# Autodesk Inventor assembly: BG401_trajan20_21
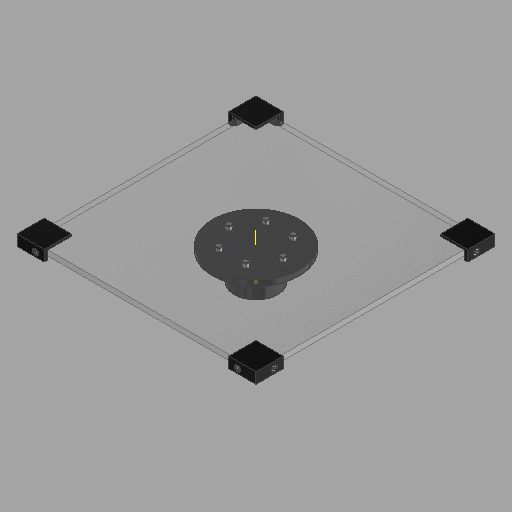
[picture p0: Inventor's stored thumbnail of the model, 512x512]
Saved by Autodesk Inventor 2022.2 (Build 262287000, 287)
## iProperties
Company: HTBLA Kaindorf
RuleStatus: InUse
Created: 2022-08-22
Part Number: BG401_trajan20_21
Project: Zeichenmaschine_v2
Material: Generisch
Description: papierplatte
Document SubType Name: Assembly
Designer: trajan20
AfterDocNew0: iProperties-Editor_aufrufen
Author: jan
Keywords: 2021
## Documents named in this file (6)
- C:\Users\jan\Documents\DrawMachine\DrawMachineConstruction\Projekt\Zeichenmaschine_v2\BG401_trajan20_21_Zeichenmaschine_v2_papierplatte.iam
- C:\Users\jan\Documents\DrawMachine\DrawMachineConstruction\Projekt\Zeichenmaschine_v2\BT403_trajan20_21_Zeichenmaschine_v2_papierplatte_plexi.ipt
- C:\Users\jan\Documents\DrawMachine\DrawMachineConstruction\Projekt\Zeichenmaschine_v2\BT406_trajan20_21_Zeichenmaschine_v2_Ecken.ipt
- C:\Users\jan\Documents\DrawMachine\DrawMachineConstruction\Projekt\Zeichenmaschine_v2\Normteile\de-DE\ISO 4762(2)\ISO 4762 - M3 x 8ISO.ipt
- C:\Users\jan\Documents\DrawMachine\DrawMachineConstruction\Projekt\Zeichenmaschine_v2\BT405_trajan20_21_Zeichenmaschine_v2_zwischenteil_stifte.ipt
- C:\Users\jan\Documents\DrawMachine\DrawMachineConstruction\Projekt\Zeichenmaschine_v2\Normteile\de-DE\ISO 2338(1)\DIN EN ISO 2338 - 5 h8 x 16.ipt
## Components (20 placed, 5 different names)
1. BT403_trajan20_21_Zeichenmaschine_v2_papierplatte_plexi:1 — Passend:1, Passend:2, Passend:3, Passend:7, Passend:8, Passend:9, Passend:10, Passend:11, Passend:12, Passend:13, Passend:14, Passend:15, Passend:28, Passend:29, Passend:30, Passend:31, Passend:32, Passend:33, Passend:34, Passend:35, Passend:36, Passend:37, Passend:38, Passend:39, Passend:40
2. BT406_trajan20_21_Zeichenmaschine_v2_Ecken:1 — Passend:1, Passend:2, Passend:4, Passend:5, Passend:6
3. ISO 4762 M3 x 8:1 — Passend:3, Passend:4
4. ISO 4762 M3 x 8:2 — Passend:5, Passend:6
5. BT406_trajan20_21_Zeichenmaschine_v2_Ecken:2 — Passend:7, Passend:8, Passend:9, Passend:16, Passend:17, Passend:18, Passend:19
6. BT406_trajan20_21_Zeichenmaschine_v2_Ecken:3 — Passend:10, Passend:11, Passend:12, Passend:24, Passend:25, Passend:26, Passend:27
7. BT406_trajan20_21_Zeichenmaschine_v2_Ecken:4 — Passend:13, Passend:14, Passend:15, Passend:20, Passend:21, Passend:22, Passend:23
8. ISO 4762 M3 x 8:3 — Passend:16, Passend:17
9. ISO 4762 M3 x 8:4 — Passend:18, Passend:19
10. ISO 4762 M3 x 8:5 — Passend:20, Passend:21
11. ISO 4762 M3 x 8:6 — Passend:22, Passend:23
12. ISO 4762 M3 x 8:7 — Passend:24, Passend:25
13. ISO 4762 M3 x 8:8 — Passend:26, Passend:27
14. BT405_trajan20_21_Zeichenmaschine_v2_zwischenteil_stifte:1 — Passend:28, Passend:41, Passend:42
15. DIN EN ISO 2338 5 h8 x 16:1 — Passend:29, Passend:30
16. DIN EN ISO 2338 5 h8 x 16:2 — Passend:31, Passend:32, Passend:42
17. DIN EN ISO 2338 5 h8 x 16:3 — Passend:33, Passend:34
18. DIN EN ISO 2338 5 h8 x 16:4 — Passend:35, Passend:36
19. DIN EN ISO 2338 5 h8 x 16:5 — Passend:37, Passend:38, Passend:41
20. DIN EN ISO 2338 5 h8 x 16:6 — Passend:39, Passend:40
## Relationships (42: Mate 42)
- Passend:1 [Mate]: BT403_trajan20_21_Zeichenmaschine_v2_papierplatte_plexi:1 ↔ BT406_trajan20_21_Zeichenmaschine_v2_Ecken:1
- Passend:2 [Mate]: BT403_trajan20_21_Zeichenmaschine_v2_papierplatte_plexi:1 ↔ BT406_trajan20_21_Zeichenmaschine_v2_Ecken:1
- Passend:3 [Mate]: BT403_trajan20_21_Zeichenmaschine_v2_papierplatte_plexi:1 ↔ ISO 4762 M3 x 8:1
- Passend:4 [Mate]: BT406_trajan20_21_Zeichenmaschine_v2_Ecken:1 ↔ ISO 4762 M3 x 8:1
- Passend:5 [Mate]: BT406_trajan20_21_Zeichenmaschine_v2_Ecken:1 ↔ ISO 4762 M3 x 8:2
- Passend:6 [Mate]: BT406_trajan20_21_Zeichenmaschine_v2_Ecken:1 ↔ ISO 4762 M3 x 8:2
- Passend:7 [Mate]: BT403_trajan20_21_Zeichenmaschine_v2_papierplatte_plexi:1 ↔ BT406_trajan20_21_Zeichenmaschine_v2_Ecken:2
- Passend:8 [Mate]: BT403_trajan20_21_Zeichenmaschine_v2_papierplatte_plexi:1 ↔ BT406_trajan20_21_Zeichenmaschine_v2_Ecken:2
- Passend:9 [Mate]: BT403_trajan20_21_Zeichenmaschine_v2_papierplatte_plexi:1 ↔ BT406_trajan20_21_Zeichenmaschine_v2_Ecken:2
- Passend:10 [Mate]: BT403_trajan20_21_Zeichenmaschine_v2_papierplatte_plexi:1 ↔ BT406_trajan20_21_Zeichenmaschine_v2_Ecken:3
- Passend:11 [Mate]: BT403_trajan20_21_Zeichenmaschine_v2_papierplatte_plexi:1 ↔ BT406_trajan20_21_Zeichenmaschine_v2_Ecken:3
- Passend:12 [Mate]: BT403_trajan20_21_Zeichenmaschine_v2_papierplatte_plexi:1 ↔ BT406_trajan20_21_Zeichenmaschine_v2_Ecken:3
- Passend:13 [Mate]: BT403_trajan20_21_Zeichenmaschine_v2_papierplatte_plexi:1 ↔ BT406_trajan20_21_Zeichenmaschine_v2_Ecken:4
- Passend:14 [Mate]: BT403_trajan20_21_Zeichenmaschine_v2_papierplatte_plexi:1 ↔ BT406_trajan20_21_Zeichenmaschine_v2_Ecken:4
- Passend:15 [Mate]: BT403_trajan20_21_Zeichenmaschine_v2_papierplatte_plexi:1 ↔ BT406_trajan20_21_Zeichenmaschine_v2_Ecken:4
- Passend:16 [Mate]: BT406_trajan20_21_Zeichenmaschine_v2_Ecken:2 ↔ ISO 4762 M3 x 8:3
- Passend:17 [Mate]: BT406_trajan20_21_Zeichenmaschine_v2_Ecken:2 ↔ ISO 4762 M3 x 8:3
- Passend:18 [Mate]: BT406_trajan20_21_Zeichenmaschine_v2_Ecken:2 ↔ ISO 4762 M3 x 8:4
- Passend:19 [Mate]: BT406_trajan20_21_Zeichenmaschine_v2_Ecken:2 ↔ ISO 4762 M3 x 8:4
- Passend:20 [Mate]: BT406_trajan20_21_Zeichenmaschine_v2_Ecken:4 ↔ ISO 4762 M3 x 8:5
- Passend:21 [Mate]: BT406_trajan20_21_Zeichenmaschine_v2_Ecken:4 ↔ ISO 4762 M3 x 8:5
- Passend:22 [Mate]: BT406_trajan20_21_Zeichenmaschine_v2_Ecken:4 ↔ ISO 4762 M3 x 8:6
- Passend:23 [Mate]: BT406_trajan20_21_Zeichenmaschine_v2_Ecken:4 ↔ ISO 4762 M3 x 8:6
- Passend:24 [Mate]: BT406_trajan20_21_Zeichenmaschine_v2_Ecken:3 ↔ ISO 4762 M3 x 8:7
- Passend:25 [Mate]: BT406_trajan20_21_Zeichenmaschine_v2_Ecken:3 ↔ ISO 4762 M3 x 8:7
- Passend:26 [Mate]: BT406_trajan20_21_Zeichenmaschine_v2_Ecken:3 ↔ ISO 4762 M3 x 8:8
- Passend:27 [Mate]: BT406_trajan20_21_Zeichenmaschine_v2_Ecken:3 ↔ ISO 4762 M3 x 8:8
- Passend:28 [Mate]: BT403_trajan20_21_Zeichenmaschine_v2_papierplatte_plexi:1 ↔ BT405_trajan20_21_Zeichenmaschine_v2_zwischenteil_stifte:1
- Passend:29 [Mate]: BT403_trajan20_21_Zeichenmaschine_v2_papierplatte_plexi:1 ↔ DIN EN ISO 2338 5 h8 x 16:1
- Passend:30 [Mate]: BT403_trajan20_21_Zeichenmaschine_v2_papierplatte_plexi:1 ↔ DIN EN ISO 2338 5 h8 x 16:1
- Passend:31 [Mate]: BT403_trajan20_21_Zeichenmaschine_v2_papierplatte_plexi:1 ↔ DIN EN ISO 2338 5 h8 x 16:2
- Passend:32 [Mate]: BT403_trajan20_21_Zeichenmaschine_v2_papierplatte_plexi:1 ↔ DIN EN ISO 2338 5 h8 x 16:2
- Passend:33 [Mate]: BT403_trajan20_21_Zeichenmaschine_v2_papierplatte_plexi:1 ↔ DIN EN ISO 2338 5 h8 x 16:3
- Passend:34 [Mate]: BT403_trajan20_21_Zeichenmaschine_v2_papierplatte_plexi:1 ↔ DIN EN ISO 2338 5 h8 x 16:3
- Passend:35 [Mate]: BT403_trajan20_21_Zeichenmaschine_v2_papierplatte_plexi:1 ↔ DIN EN ISO 2338 5 h8 x 16:4
- Passend:36 [Mate]: BT403_trajan20_21_Zeichenmaschine_v2_papierplatte_plexi:1 ↔ DIN EN ISO 2338 5 h8 x 16:4
- Passend:37 [Mate]: BT403_trajan20_21_Zeichenmaschine_v2_papierplatte_plexi:1 ↔ DIN EN ISO 2338 5 h8 x 16:5
- Passend:38 [Mate]: BT403_trajan20_21_Zeichenmaschine_v2_papierplatte_plexi:1 ↔ DIN EN ISO 2338 5 h8 x 16:5
- Passend:39 [Mate]: BT403_trajan20_21_Zeichenmaschine_v2_papierplatte_plexi:1 ↔ DIN EN ISO 2338 5 h8 x 16:6
- Passend:40 [Mate]: BT403_trajan20_21_Zeichenmaschine_v2_papierplatte_plexi:1 ↔ DIN EN ISO 2338 5 h8 x 16:6
- Passend:41 [Mate]: BT405_trajan20_21_Zeichenmaschine_v2_zwischenteil_stifte:1 ↔ DIN EN ISO 2338 5 h8 x 16:5
- Passend:42 [Mate]: BT405_trajan20_21_Zeichenmaschine_v2_zwischenteil_stifte:1 ↔ DIN EN ISO 2338 5 h8 x 16:2
